# Autodesk Inventor assembly: Fahrbasis
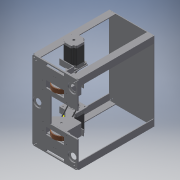
[picture p0: Inventor's stored thumbnail of the model, 180x180]
Saved by Autodesk Inventor 2017 (Build 210142000, 142)
## iProperties
Part Number: Fahrbasis
Material: Generisch
Document SubType Name: Assembly
Designer: Dima
Author: Dima
## Documents named in this file (13)
- C:\Users\Dima\Desktop\Projektarbeit Roboteam\Entwurf Roboplatform\Fahrbasis.iam
- C:\Users\Dima\Desktop\Projektarbeit Roboteam\Entwurf Roboplatform\Grundplatte.ipt
- C:\Users\Dima\Desktop\Projektarbeit Roboteam\Entwurf Roboplatform\Motorhalterung_Links.ipt
- C:\Users\Dima\Desktop\Projektarbeit Roboteam\Entwurf Roboplatform\Motorhalterung_Rechts.ipt
- C:\Users\Dima\Desktop\Projektarbeit Roboteam\Entwurf Roboplatform\Radkasten_Links.ipt
- C:\Users\Dima\Desktop\Projektarbeit Roboteam\Entwurf Roboplatform\Radkasten_Rechts.ipt
- C:\Users\Dima\Desktop\Projektarbeit Roboteam\Entwurf Roboplatform\Rad.ipt
- C:\Users\Dima\Desktop\Projektarbeit Roboteam\Entwurf Roboplatform\16222000.ipt
- C:\Users\Dima\Desktop\Projektarbeit Roboteam\Entwurf Roboplatform\QSH6018-86-28.iam
- C:\Users\Dima\Desktop\Projektarbeit Roboteam\Entwurf Roboplatform\Fahrbasis\Konstruktions-Assistent\Übertragung des Zahnriemens1.iam
- C:\Users\Dima\Desktop\Projektarbeit Roboteam\Entwurf Roboplatform\Fahrbasis\Konstruktions-Assistent\Übertragung des Zahnriemens2.iam
- C:\Users\Dima\Desktop\Projektarbeit Roboteam\Entwurf Roboplatform\Schiene.ipt
- C:\Users\Dima\Desktop\Projektarbeit Roboteam\Entwurf Roboplatform\Deckplatte.ipt
## Components (20 placed, 11 different names)
1. Grundplatte:1 — Fluchtend:1, Fluchtend:2, Fluchtend:3, Passend:1, Passend:2, Passend:3, Passend:5, Passend:6, Passend:7, Passend:21, Passend:22, Passend:23, Passend:24, Fluchtend:14, Fluchtend:15, Fluchtend:16, Fluchtend:17, Fluchtend:18, Fluchtend:19, Fluchtend:20, Fluchtend:21
2. Motorhalterung_Links:1 — Passend:8, Fluchtend:6, Fluchtend:7, Passend:9, Passend:11, Winkel:1
3. Motorhalterung_Rechts:1 — Passend:4, Fluchtend:4, Fluchtend:5, Passend:10, Passend:12, Winkel:2
4. Radkasten_Rechts:1 — Passend:1, Passend:2, Passend:3, Passend:4, Fluchtend:4, Fluchtend:5, Passend:19
5. Radkasten_Links:1 — Passend:5, Passend:6, Passend:7, Passend:8, Fluchtend:6, Fluchtend:7, Passend:20
6. Rad:1 — Passend:15, Passend:16
7. Rad:2 — Passend:17, Passend:18
8. 16222000:1 — Passend:14, Fluchtend:9, Fluchtend:10, Drehung:2, Fluchtend:13
9. 16222000:2 — Passend:15, Passend:16, Fluchtend:10, Passend:19, Drehung:2
10. 16222000:3 — Passend:13, Fluchtend:8, Fluchtend:11, Fluchtend:12, Drehung:1
11. 16222000:4 — Passend:17, Passend:18, Fluchtend:11, Passend:20, Drehung:1
12. QSH6018-86-28:1 [sub-assembly] — Passend:10, Passend:12, Winkel:2, Passend:14, Fluchtend:9
13. QSH6018-86-28:2 [sub-assembly] — Passend:9, Passend:11, Winkel:1, Passend:13, Fluchtend:8
14. Übertragung des Zahnriemens:1 [sub-assembly]
15. Übertragung des Zahnriemens:2 [sub-assembly]
16. Schiene:1 — Passend:21, Fluchtend:20, Fluchtend:21, Fluchtend:22, Fluchtend:23
17. Schiene:2 — Passend:22, Passend:25, Fluchtend:16, Fluchtend:17
18. Schiene:3 — Passend:23, Fluchtend:18, Fluchtend:19
19. Schiene:4 — Passend:24, Fluchtend:14, Fluchtend:15
20. Deckplatte:1 — Passend:25, Fluchtend:22, Fluchtend:23
## Relationships (52: Mate 25, Flush 23, Angle 2, RelateRotation 2)
- Fluchtend:1 [Flush]: Grundplatte:1
- Fluchtend:2 [Flush]: Grundplatte:1
- Fluchtend:3 [Flush]: Grundplatte:1
- Passend:1 [Mate]: Grundplatte:1 ↔ Radkasten_Rechts:1
- Passend:2 [Mate]: Grundplatte:1 ↔ Radkasten_Rechts:1
- Passend:3 [Mate]: Grundplatte:1 ↔ Radkasten_Rechts:1
- Passend:4 [Mate]: Motorhalterung_Rechts:1 ↔ Radkasten_Rechts:1
- Fluchtend:4 [Flush]: Motorhalterung_Rechts:1 ↔ Radkasten_Rechts:1
- Fluchtend:5 [Flush] (6 mm): Motorhalterung_Rechts:1 ↔ Radkasten_Rechts:1
- Passend:5 [Mate]: Grundplatte:1 ↔ Radkasten_Links:1
- Passend:6 [Mate]: Grundplatte:1 ↔ Radkasten_Links:1
- Passend:7 [Mate]: Grundplatte:1 ↔ Radkasten_Links:1
- Passend:8 [Mate]: Motorhalterung_Links:1 ↔ Radkasten_Links:1
- Fluchtend:6 [Flush]: Motorhalterung_Links:1 ↔ Radkasten_Links:1
- Fluchtend:7 [Flush] (6 mm): Motorhalterung_Links:1 ↔ Radkasten_Links:1
- Passend:9 [Mate]: Motorhalterung_Links:1 ↔ QSH6018-86-28:2
- Passend:10 [Mate]: Motorhalterung_Rechts:1 ↔ QSH6018-86-28:1
- Passend:11 [Mate]: Motorhalterung_Links:1 ↔ QSH6018-86-28:2
- Passend:12 [Mate]: Motorhalterung_Rechts:1 ↔ QSH6018-86-28:1
- Winkel:1 [Angle] (0 deg): Motorhalterung_Links:1 ↔ QSH6018-86-28:2
- Winkel:2 [Angle] (0 deg): Motorhalterung_Rechts:1 ↔ QSH6018-86-28:1
- Passend:13 [Mate]: 16222000:3 ↔ QSH6018-86-28:2
- Passend:14 [Mate]: 16222000:1 ↔ QSH6018-86-28:1
- Fluchtend:8 [Flush]: 16222000:3 ↔ QSH6018-86-28:2
- Fluchtend:9 [Flush]: 16222000:1 ↔ QSH6018-86-28:1
- Passend:15 [Mate]: Rad:1 ↔ 16222000:2
- Passend:16 [Mate]: Rad:1 ↔ 16222000:2
- Passend:17 [Mate]: Rad:2 ↔ 16222000:4
- Passend:18 [Mate]: Rad:2 ↔ 16222000:4
- Fluchtend:10 [Flush]: 16222000:1 ↔ 16222000:2
- Passend:19 [Mate]: Radkasten_Rechts:1 ↔ 16222000:2
- Fluchtend:11 [Flush]: 16222000:3 ↔ 16222000:4
- Passend:20 [Mate]: Radkasten_Links:1 ↔ 16222000:4
- Fluchtend:12 [Flush] (6.25 mm): 16222000:3
- Drehung:1 [RelateRotation] (1 ul): 16222000:3 ↔ 16222000:4
- Drehung:2 [RelateRotation] (1 ul): 16222000:1 ↔ 16222000:2
- Fluchtend:13 [Flush] (6.5 mm): 16222000:1
- Passend:21 [Mate]: Grundplatte:1 ↔ Schiene:1
- Passend:22 [Mate]: Grundplatte:1 ↔ Schiene:2
- Passend:23 [Mate]: Grundplatte:1 ↔ Schiene:3
- Passend:24 [Mate]: Grundplatte:1 ↔ Schiene:4
- Passend:25 [Mate]: Schiene:2 ↔ Deckplatte:1
- Fluchtend:14 [Flush]: Grundplatte:1 ↔ Schiene:4
- Fluchtend:15 [Flush]: Grundplatte:1 ↔ Schiene:4
- Fluchtend:16 [Flush]: Grundplatte:1 ↔ Schiene:2
- Fluchtend:17 [Flush]: Grundplatte:1 ↔ Schiene:2
- Fluchtend:18 [Flush]: Grundplatte:1 ↔ Schiene:3
- Fluchtend:19 [Flush]: Grundplatte:1 ↔ Schiene:3
- Fluchtend:20 [Flush]: Grundplatte:1 ↔ Schiene:1
- Fluchtend:21 [Flush]: Grundplatte:1 ↔ Schiene:1
- Fluchtend:22 [Flush]: Schiene:1 ↔ Deckplatte:1
- Fluchtend:23 [Flush]: Schiene:1 ↔ Deckplatte:1
